# Autodesk Inventor assembly: Klapp-Baugruppe_vorn
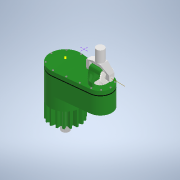
[picture p0: Inventor's stored thumbnail of the model, 180x180]
Saved by Autodesk Inventor 2021 (Build 250183000, 183)
## iProperties
Created: 2021-01-12
Part Number: Klapp-Baugruppe_vorn
Document SubType Name: Assembly
Designer: Jaro Machnow
Author: Jaro Machnow
## Documents named in this file (16)
- C:\Users\Jaro Machnow\Documents\Vault\Gruppen\Gruppe 2\Entwurf\Amphibienfahrzeug\Wechsel zwischen Land und Wasser\Wechselmechanik\Klappmechanismus2\Klapp-Baugruppe_vorn.iam
- C:\Users\Jaro Machnow\Documents\Vault\Gruppen\Gruppe 2\Entwurf\Amphibienfahrzeug\Wechsel zwischen Land und Wasser\Wechselmechanik\Klappmechanismus\Klapphülle.ipt
- C:\Users\Jaro Machnow\Documents\Vault\Gruppen\Gruppe 2\Entwurf\Amphibienfahrzeug\Wechsel zwischen Land und Wasser\Wechselmechanik\Klappmechanismus\Klapp_Welle_zur_Karosserie.ipt
- C:\Users\Jaro Machnow\Documents\Vault\Gruppen\Gruppe 2\Entwurf\Amphibienfahrzeug\Wechsel zwischen Land und Wasser\Wechselmechanik\Klappmechanismus\Klapp_ Kraftübertragung mit Keilriemen.iam
- C:\Users\Jaro Machnow\Documents\Vault\Gruppen\Gruppe 2\Entwurf\Amphibienfahrzeug\Wechsel zwischen Land und Wasser\Wechselmechanik\Klappmechanismus\Klapp_Lager.iam
- C:\Users\Jaro Machnow\Documents\Vault\Gruppen\Gruppe 2\Entwurf\Amphibienfahrzeug\Wechsel zwischen Land und Wasser\Wechselmechanik\Klappmechanismus\Keilverbindung1.iam
- C:\Users\Jaro Machnow\Documents\Vault\Gruppen\Gruppe 2\Entwurf\Amphibienfahrzeug\Wechsel zwischen Land und Wasser\Wechselmechanik\Klappmechanismus\Klapp_Dichtungsgummi.ipt
- C:\Users\Jaro Machnow\Documents\Vault\Gruppen\Gruppe 2\Entwurf\Amphibienfahrzeug\Betrieb an Land\Lenkung\Lenkung_Baugruppe.iam
- C:\Users\Jaro Machnow\Documents\Vault\Gruppen\Gruppe 2\Entwurf\Amphibienfahrzeug\Wechsel zwischen Land und Wasser\Wechselmechanik\Klappmechanismus2\Klapp_Vorn_Abdeckung.ipt
- C:\Users\Jaro Machnow\Documents\Vault\Gruppen\Gruppe 2\Entwurf\Amphibienfahrzeug\Wechsel zwischen Land und Wasser\Wechselmechanik\Klappmechanismus2\Klapp-Baugruppe\Konstruktions-Assistent\Keilverbindung4.iam
- C:\Users\Jaro Machnow\Documents\Vault\Gruppen\Gruppe 2\Entwurf\Amphibienfahrzeug\Betrieb an Land\Lenkung\Lenkung_Lenkteil_zum_Rad.ipt
- C:\Users\Jaro Machnow\Documents\Vault\Gruppen\Gruppe 2\Entwurf\Amphibienfahrzeug\Wechsel zwischen Land und Wasser\Wechselmechanik\Klappmechanismus2\Klapp-Vorn_Welle_Lenkung.ipt
- C:\Users\Jaro Machnow\Documents\Vault\Gruppen\Gruppe 2\Entwurf\Amphibienfahrzeug\Wechsel zwischen Land und Wasser\Wechselmechanik\Klappmechanismus2\Klapp_Vorn_Welle_Rad.ipt
- C:\Users\Jaro Machnow\Documents\Vault\Gruppen\Gruppe 2\Entwurf\Amphibienfahrzeug\Wechsel zwischen Land und Wasser\Wechselmechanik\Klappmechanismus2\Klapp-Baugruppe\Konstruktions-Assistent\Keilverbindung5.iam
- C:\Users\Jaro Machnow\Documents\Vault\Gruppen\Gruppe 2\Entwurf\Amphibienfahrzeug\Wechsel zwischen Land und Wasser\Wechselmechanik\Klappmechanismus2\Klapp-Baugruppe\Konstruktions-Assistent\Keilverbindung6.iam
- C:\Users\Jaro Machnow\Documents\Inventor\Content Center Files\R2021\de-DE\DIN 84\DIN 84 - M1 x 10.ipt
## Components (31 placed, 10 different names)
1. Welle:1 — Passend:1, Passend:5, Fluchtend:6, Passend:10, Passend:11, Passend:12, Winkel:2, Passend:71, Fluchtend:27, Winkel:37, Passend:114
2. Kraftübertragung mit Keilriemen:1 [sub-assembly] — Passend:1, Passend:10, Winkel:2, Passend:61, Passend:66, Winkel:21
3. Lager:1 [sub-assembly] — Passend:5, Fluchtend:6, Passend:21
4. Lager:2 [sub-assembly] — Passend:64, Passend:65
5. Lager:3 [sub-assembly] — Passend:11, Passend:12
6. Keilverbindung:1 [sub-assembly] — Fluchtend:27, Winkel:37, Passend:114
7. Lager:4 [sub-assembly] — Passend:62, Passend:63
8. Klapphülle:1 — Passend:21, Passend:22, Passend:23, Passend:24, Passend:33, Passend:34, Passend:71
9. Klapp_Dichtungsgummi:1 — Passend:22, Passend:23, Passend:24, Passend:32
10. Lenkung_Baugruppe:1 [sub-assembly] — Passend:56, Winkel:19, Winkel:23, Passend:74
11. Klapp_Vorn_Abdeckung:1 — Passend:32, Passend:33, Passend:34, Passend:55, Passend:70, Passend:75, Passend:76, Passend:77, Passend:78, Passend:79, Passend:80, Passend:81, Passend:82, Passend:83, Passend:84, Passend:85, Passend:86, Passend:87, Passend:88, Passend:89, Passend:90, Passend:91, Passend:92, Passend:93, Passend:94, Passend:95, Passend:96, Passend:97, Passend:98, Passend:99, Passend:100, Passend:101, Passend:102, Passend:115
12. Lenkung_Lenkteil_zum_Rad:1 — Passend:115, Passend:116
13. Welle:1 — Passend:55, Passend:56, Winkel:19, Fluchtend:24, Winkel:34, Passend:111, Passend:116
14. Keilverbindung:4 [sub-assembly] — Fluchtend:24, Winkel:34, Passend:111
15. Welle:1 — Passend:61, Passend:62, Passend:63, Passend:64, Passend:65, Passend:66, Winkel:21, Winkel:23, Passend:70, Passend:74, Fluchtend:26, Winkel:36, Passend:113, Fluchtend:28, Winkel:38, Passend:117
16. Keilverbindung:5 [sub-assembly] — Fluchtend:28, Winkel:38, Passend:117
17. Keilverbindung:6 [sub-assembly] — Fluchtend:26, Winkel:36, Passend:113
18. DIN 84 - ersetzt durch DIN EN ISO 1207 M1 x 10:1 — Passend:75, Passend:76
19. DIN 84 - ersetzt durch DIN EN ISO 1207 M1 x 10:2 — Passend:77, Passend:78
20. DIN 84 - ersetzt durch DIN EN ISO 1207 M1 x 10:3 — Passend:79, Passend:80
21. DIN 84 - ersetzt durch DIN EN ISO 1207 M1 x 10:4 — Passend:81, Passend:82
22. DIN 84 - ersetzt durch DIN EN ISO 1207 M1 x 10:5 — Passend:83, Passend:84
23. DIN 84 - ersetzt durch DIN EN ISO 1207 M1 x 10:6 — Passend:85, Passend:86
24. DIN 84 - ersetzt durch DIN EN ISO 1207 M1 x 10:7 — Passend:87, Passend:88
25. DIN 84 - ersetzt durch DIN EN ISO 1207 M1 x 10:8 — Passend:89, Passend:90
26. DIN 84 - ersetzt durch DIN EN ISO 1207 M1 x 10:9 — Passend:91, Passend:92
27. DIN 84 - ersetzt durch DIN EN ISO 1207 M1 x 10:10 — Passend:93, Passend:94
28. DIN 84 - ersetzt durch DIN EN ISO 1207 M1 x 10:11 — Passend:95, Passend:96
29. DIN 84 - ersetzt durch DIN EN ISO 1207 M1 x 10:12 — Passend:97, Passend:98
30. DIN 84 - ersetzt durch DIN EN ISO 1207 M1 x 10:13 — Passend:99, Passend:100
31. DIN 84 - ersetzt durch DIN EN ISO 1207 M1 x 10:14 — Passend:101, Passend:102
## Relationships (70: Mate 57, Angle 8, Flush 5)
- Passend:1 [Mate]: Welle:1 ↔ Kraftübertragung mit Keilriemen:1
- Passend:5 [Mate]: Welle:1 ↔ Lager:1
- Fluchtend:6 [Flush]: Welle:1 ↔ Lager:1
- Passend:10 [Mate]: Welle:1 ↔ Kraftübertragung mit Keilriemen:1
- Passend:11 [Mate]: Welle:1 ↔ Lager:3
- Passend:12 [Mate]: Welle:1 ↔ Lager:3
- Winkel:2 [Angle] (174.2383 deg): Welle:1 ↔ Kraftübertragung mit Keilriemen:1
- Passend:21 [Mate]: Lager:1 ↔ Klapphülle:1
- Passend:22 [Mate]: Klapphülle:1 ↔ Klapp_Dichtungsgummi:1
- Passend:23 [Mate]: Klapphülle:1 ↔ Klapp_Dichtungsgummi:1
- Passend:24 [Mate]: Klapphülle:1 ↔ Klapp_Dichtungsgummi:1
- Passend:32 [Mate]: Klapp_Dichtungsgummi:1 ↔ Klapp_Vorn_Abdeckung:1
- Passend:33 [Mate]: Klapphülle:1 ↔ Klapp_Vorn_Abdeckung:1
- Passend:34 [Mate]: Klapphülle:1 ↔ Klapp_Vorn_Abdeckung:1
- Passend:55 [Mate]: Klapp_Vorn_Abdeckung:1 ↔ Welle:1
- Passend:56 [Mate]: Lenkung_Baugruppe:1 ↔ Welle:1
- Winkel:19 [Angle] (173.4856 deg): Lenkung_Baugruppe:1 ↔ Welle:1
- Passend:61 [Mate]: Kraftübertragung mit Keilriemen:1 ↔ Welle:1
- Passend:62 [Mate]: Lager:4 ↔ Welle:1
- Passend:63 [Mate]: Lager:4 ↔ Welle:1
- Passend:64 [Mate]: Lager:2 ↔ Welle:1
- Passend:65 [Mate]: Lager:2 ↔ Welle:1
- Passend:66 [Mate]: Kraftübertragung mit Keilriemen:1 ↔ Welle:1
- Winkel:21 [Angle] (141.9438 deg): Kraftübertragung mit Keilriemen:1 ↔ Welle:1
- Winkel:23 [Angle] (15.1609 deg): Lenkung_Baugruppe:1 ↔ Welle:1
- Passend:70 [Mate] (0.064 mm): Klapp_Vorn_Abdeckung:1 ↔ Welle:1
- Passend:71 [Mate] (0.021 mm): Welle:1 ↔ Klapphülle:1
- Passend:74 [Mate]: Lenkung_Baugruppe:1 ↔ Welle:1
- Passend:75 [Mate]: Klapp_Vorn_Abdeckung:1 ↔ DIN 84 - ersetzt durch DIN EN ISO 1207 M1 x 10:1
- Passend:76 [Mate]: Klapp_Vorn_Abdeckung:1 ↔ DIN 84 - ersetzt durch DIN EN ISO 1207 M1 x 10:1
- Passend:77 [Mate]: Klapp_Vorn_Abdeckung:1 ↔ DIN 84 - ersetzt durch DIN EN ISO 1207 M1 x 10:2
- Passend:78 [Mate]: Klapp_Vorn_Abdeckung:1 ↔ DIN 84 - ersetzt durch DIN EN ISO 1207 M1 x 10:2
- Passend:79 [Mate]: Klapp_Vorn_Abdeckung:1 ↔ DIN 84 - ersetzt durch DIN EN ISO 1207 M1 x 10:3
- Passend:80 [Mate]: Klapp_Vorn_Abdeckung:1 ↔ DIN 84 - ersetzt durch DIN EN ISO 1207 M1 x 10:3
- Passend:81 [Mate]: Klapp_Vorn_Abdeckung:1 ↔ DIN 84 - ersetzt durch DIN EN ISO 1207 M1 x 10:4
- Passend:82 [Mate]: Klapp_Vorn_Abdeckung:1 ↔ DIN 84 - ersetzt durch DIN EN ISO 1207 M1 x 10:4
- Passend:83 [Mate]: Klapp_Vorn_Abdeckung:1 ↔ DIN 84 - ersetzt durch DIN EN ISO 1207 M1 x 10:5
- Passend:84 [Mate]: Klapp_Vorn_Abdeckung:1 ↔ DIN 84 - ersetzt durch DIN EN ISO 1207 M1 x 10:5
- Passend:85 [Mate]: Klapp_Vorn_Abdeckung:1 ↔ DIN 84 - ersetzt durch DIN EN ISO 1207 M1 x 10:6
- Passend:86 [Mate]: Klapp_Vorn_Abdeckung:1 ↔ DIN 84 - ersetzt durch DIN EN ISO 1207 M1 x 10:6
- Passend:87 [Mate]: Klapp_Vorn_Abdeckung:1 ↔ DIN 84 - ersetzt durch DIN EN ISO 1207 M1 x 10:7
- Passend:88 [Mate]: Klapp_Vorn_Abdeckung:1 ↔ DIN 84 - ersetzt durch DIN EN ISO 1207 M1 x 10:7
- Passend:89 [Mate]: Klapp_Vorn_Abdeckung:1 ↔ DIN 84 - ersetzt durch DIN EN ISO 1207 M1 x 10:8
- Passend:90 [Mate]: Klapp_Vorn_Abdeckung:1 ↔ DIN 84 - ersetzt durch DIN EN ISO 1207 M1 x 10:8
- Passend:91 [Mate]: Klapp_Vorn_Abdeckung:1 ↔ DIN 84 - ersetzt durch DIN EN ISO 1207 M1 x 10:9
- Passend:92 [Mate]: Klapp_Vorn_Abdeckung:1 ↔ DIN 84 - ersetzt durch DIN EN ISO 1207 M1 x 10:9
- Passend:93 [Mate]: Klapp_Vorn_Abdeckung:1 ↔ DIN 84 - ersetzt durch DIN EN ISO 1207 M1 x 10:10
- Passend:94 [Mate]: Klapp_Vorn_Abdeckung:1 ↔ DIN 84 - ersetzt durch DIN EN ISO 1207 M1 x 10:10
- Passend:95 [Mate]: Klapp_Vorn_Abdeckung:1 ↔ DIN 84 - ersetzt durch DIN EN ISO 1207 M1 x 10:11
- Passend:96 [Mate]: Klapp_Vorn_Abdeckung:1 ↔ DIN 84 - ersetzt durch DIN EN ISO 1207 M1 x 10:11
- Passend:97 [Mate]: Klapp_Vorn_Abdeckung:1 ↔ DIN 84 - ersetzt durch DIN EN ISO 1207 M1 x 10:12
- Passend:98 [Mate]: Klapp_Vorn_Abdeckung:1 ↔ DIN 84 - ersetzt durch DIN EN ISO 1207 M1 x 10:12
- Passend:99 [Mate]: Klapp_Vorn_Abdeckung:1 ↔ DIN 84 - ersetzt durch DIN EN ISO 1207 M1 x 10:13
- Passend:100 [Mate]: Klapp_Vorn_Abdeckung:1 ↔ DIN 84 - ersetzt durch DIN EN ISO 1207 M1 x 10:13
- Passend:101 [Mate]: Klapp_Vorn_Abdeckung:1 ↔ DIN 84 - ersetzt durch DIN EN ISO 1207 M1 x 10:14
- Passend:102 [Mate]: Klapp_Vorn_Abdeckung:1 ↔ DIN 84 - ersetzt durch DIN EN ISO 1207 M1 x 10:14
- Fluchtend:24 [Flush] (0.371 mm): Welle:1 ↔ Keilverbindung:4
- Winkel:34 [Angle] (0 deg): Welle:1 ↔ Keilverbindung:4
- Passend:111 [Mate]: Welle:1 ↔ Keilverbindung:4
- Fluchtend:26 [Flush] (0.0883 mm): Welle:1 ↔ Keilverbindung:6
- Winkel:36 [Angle] (50 deg): Welle:1 ↔ Keilverbindung:6
- Passend:113 [Mate]: Welle:1 ↔ Keilverbindung:6
- Fluchtend:27 [Flush] (1.0188 mm): Welle:1 ↔ Keilverbindung:1
- Winkel:37 [Angle] (45 deg): Welle:1 ↔ Keilverbindung:1
- Passend:114 [Mate]: Welle:1 ↔ Keilverbindung:1
- Passend:115 [Mate]: Klapp_Vorn_Abdeckung:1 ↔ Lenkung_Lenkteil_zum_Rad:1
- Passend:116 [Mate]: Lenkung_Lenkteil_zum_Rad:1 ↔ Welle:1
- Fluchtend:28 [Flush] (6.7781 mm): Welle:1 ↔ Keilverbindung:5
- Winkel:38 [Angle] (325 deg): Welle:1 ↔ Keilverbindung:5
- Passend:117 [Mate]: Welle:1 ↔ Keilverbindung:5
